# Autodesk Inventor assembly: tau2
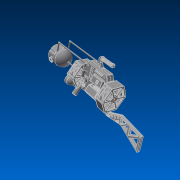
[picture p0: Inventor's stored thumbnail of the model, 180x180]
Saved by Autodesk Inventor 2020.4 (Build 244396010, 396A)
## iProperties
Created: 2022-09-08
Part Number: tau2
Document SubType Name: Assembly
Designer: Val
Author: Val
## Documents named in this file (22)
- C:\Users\Val\Desktop\tau\Tau.iam
- C:\Users\Val\Desktop\tau\external\TopHandle.ipt
- C:\Users\Val\Desktop\tau\Body2.ipt
- C:\Users\Val\Desktop\tau\Body2_MIR.ipt
- C:\Users\Val\Desktop\tau\external\FlowMeter.ipt
- C:\Users\Val\Desktop\tau\external\SideHandle.ipt
- C:\Users\Val\Desktop\tau\external\SideHandleBase.ipt
- C:\Users\Val\Desktop\tau\HexCoil.ipt
- C:\Users\Val\Desktop\tau\CoilCover.ipt
- C:\Users\Val\Desktop\tau\Stock.ipt
- C:\Users\Val\Desktop\tau\Stock_MIR.ipt
- C:\Users\Val\Desktop\tau\HoseConnector.ipt
- C:\Users\Val\Desktop\tau\BatteryCover.ipt
- C:\Users\Val\Desktop\tau\BatteryCoverLid.ipt
- C:\Users\Val\Desktop\tau\muzzle.ipt
- C:\Users\Val\Desktop\tau\MuzzleEndBall.ipt
- C:\Users\Val\Desktop\tau\MuzzleEndTube.ipt
- C:\Users\Val\Desktop\tau\ToroidalCore.ipt
- C:\Users\Val\Desktop\tau\MuzzleWireProtector.ipt
- C:\Users\Val\Desktop\tau\TopPipe.ipt
- C:\Users\Val\Desktop\tau\TopPipe_MIR.ipt
- C:\Users\Val\Desktop\tau\external\CO2Cartridge16g.ipt
## Components (29 placed, 21 different names)
1. TopHandle:1 — Mate:2
2. Body2:1 — Mate:1, Mate:2, Mate:3, Mate:4, Mate:5, Flush:3, Mate:6, Flush:4, Mate:15, Mate:26, Mate:30, Flush:35, Mate:37, Mate:38, Mate:47
3. Body2_MIR:1 — Mate:5, Flush:3, Flush:4
4. FlowMeter:1 — Mate:3, Mate:4, Mate:6
5. SideHandle:1 — Mate:7
6. SideHandleBase:1 — Mate:7
7. HexCoil:1 — Mate:13, Mate:15, Flush:6, Flush:7, Mate:27, Flush:10, Flush:11, Mate:31, Flush:12, Flush:13, Flush:37, Angle:1, Angle:2, Flush:48
8. HexCoil:2 — Flush:6, Flush:7, Mate:22, Flush:8, Mate:24, Flush:9, Mate:25, Mate:32, Flush:35
9. CoilCover:1 — Mate:22, Flush:8, Mate:25, Mate:45
10. CoilCover:2 — Mate:24, Flush:9, Mate:26
11. CoilCover:3 — Mate:31, Flush:12, Flush:13, Flush:36, Mate:33
12. CoilCover:4 — Mate:27, Flush:10, Flush:11, Mate:30
13. Stock:1 — Flush:34, Mate:32
14. Stock_MIR:1
15. HoseConnector:1 — Flush:36, Mate:33, Flush:37
16. BatteryCover:1 — Flush:38, Flush:39, Flush:44, Flush:45
17. BatteryCover:2 — Flush:38, Mate:35, Flush:40, Flush:41
18. BatteryCover:3 — Flush:39, Mate:36, Flush:42, Flush:43, Mate:39, Flush:46, Flush:47
19. BatteryCoverLid:1 — Mate:35, Flush:40, Flush:41, Mate:36, Flush:42, Flush:43, Flush:44, Flush:45, Mate:37, Mate:38
20. BatteryCoverLid:2 — Mate:39, Flush:46, Flush:47
21. muzzle:1 — Mate:42, Mate:46
22. MuzzleEndBall:1 — Mate:43, Mate:44, Mate:48
23. MuzzleEndTube:1 — Mate:42, Mate:43, Angle:1, Angle:2, Mate:44, Mate:48
24. ToroidalCore:1 — Mate:46
25. ToroidalCore:2 — Mate:45
26. MuzzleWireProtector:1
27. TopPipe:1 — Mate:47
28. TopPipe_MIR:1
29. CO2Cartridge16g:1 — Flush:48
## Relationships (58: Mate 30, Flush 25, Angle 2, Symmetry 1)
- Symmetry:1
- Mate:1: Body2:1
- Mate:2: TopHandle:1 ↔ Body2:1
- Mate:3: Body2:1 ↔ FlowMeter:1
- Mate:4: Body2:1 ↔ FlowMeter:1
- Mate:5: Body2:1 ↔ Body2_MIR:1
- Flush:3: Body2:1 ↔ Body2_MIR:1
- Mate:6: Body2:1 ↔ FlowMeter:1
- Flush:4: Body2:1 ↔ Body2_MIR:1
- Mate:7: SideHandle:1 ↔ SideHandleBase:1
- Mate:13: HexCoil:1
- Mate:15: Body2:1 ↔ HexCoil:1
- Flush:6: HexCoil:1 ↔ HexCoil:2
- Flush:7: HexCoil:1 ↔ HexCoil:2
- Mate:22: HexCoil:2 ↔ CoilCover:1
- Flush:8: HexCoil:2 ↔ CoilCover:1
- Mate:24: HexCoil:2 ↔ CoilCover:2
- Flush:9: HexCoil:2 ↔ CoilCover:2
- Mate:25: HexCoil:2 ↔ CoilCover:1
- Mate:26: Body2:1 ↔ CoilCover:2
- Mate:27: HexCoil:1 ↔ CoilCover:4
- Flush:10: HexCoil:1 ↔ CoilCover:4
- Flush:11: HexCoil:1 ↔ CoilCover:4
- Mate:30: Body2:1 ↔ CoilCover:4
- Mate:31: HexCoil:1 ↔ CoilCover:3
- Flush:12: HexCoil:1 ↔ CoilCover:3
- Flush:13: HexCoil:1 ↔ CoilCover:3
- Flush:34: Stock:1
- Mate:32: HexCoil:2 ↔ Stock:1
- Flush:35: Body2:1 ↔ HexCoil:2
- Flush:36: CoilCover:3 ↔ HoseConnector:1
- Mate:33: CoilCover:3 ↔ HoseConnector:1
- Flush:37: HexCoil:1 ↔ HoseConnector:1
- Flush:38: BatteryCover:1 ↔ BatteryCover:2
- Flush:39: BatteryCover:1 ↔ BatteryCover:3
- Mate:35: BatteryCover:2 ↔ BatteryCoverLid:1
- Flush:40: BatteryCover:2 ↔ BatteryCoverLid:1
- Flush:41: BatteryCover:2 ↔ BatteryCoverLid:1
- Mate:36: BatteryCover:3 ↔ BatteryCoverLid:1
- Flush:42: BatteryCover:3 ↔ BatteryCoverLid:1
- Flush:43: BatteryCover:3 ↔ BatteryCoverLid:1
- Flush:44: BatteryCover:1 ↔ BatteryCoverLid:1
- Flush:45: BatteryCover:1 ↔ BatteryCoverLid:1
- Mate:37: Body2:1 ↔ BatteryCoverLid:1
- Mate:38: Body2:1 ↔ BatteryCoverLid:1
- Mate:39: BatteryCover:3 ↔ BatteryCoverLid:2
- Flush:46: BatteryCover:3 ↔ BatteryCoverLid:2
- Flush:47: BatteryCover:3 ↔ BatteryCoverLid:2
- Mate:42: muzzle:1 ↔ MuzzleEndTube:1
- Mate:43: MuzzleEndBall:1 ↔ MuzzleEndTube:1
- Angle:1 (0 deg): HexCoil:1 ↔ MuzzleEndTube:1
- Angle:2 (0 deg): HexCoil:1 ↔ MuzzleEndTube:1
- Mate:44: MuzzleEndBall:1 ↔ MuzzleEndTube:1
- Mate:45: CoilCover:1 ↔ ToroidalCore:2
- Mate:46: muzzle:1 ↔ ToroidalCore:1
- Mate:47: Body2:1 ↔ TopPipe:1
- Mate:48: MuzzleEndBall:1 ↔ MuzzleEndTube:1
- Flush:48: HexCoil:1 ↔ CO2Cartridge16g:1
